# Autodesk Inventor assembly: ElectronicsHousing
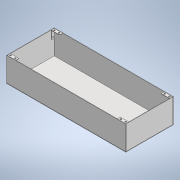
[picture p0: Inventor's stored thumbnail of the model, 180x180]
Saved by Autodesk Inventor 2020 (Build 240168000, 168)
## iProperties
Created: 2021-11-12
Part Number: ElectronicsHousing
Document SubType Name: Assembly
Designer: 17185
Author: 17185
## Documents named in this file (3)
- C:\Users\17185\Desktop\chassis draft\ElectronicsHousing\ElectronicsHousing.iam
- C:\Users\17185\Desktop\chassis draft\ElectronicsHousing\ElectronicsCasing.iam
- C:\Users\17185\Desktop\chassis draft\CornerBrace.ipt
## Components (5 placed, 2 different names)
1. ElectronicsCasing:1 [sub-assembly] — Mate:1, Mate:2, Flush:2, Mate:3, Mate:4, Mate:5, Mate:6, Mate:7, Flush:4, Mate:8
2. CornerBrace:1 — Flush:3, Mate:7, Mate:8
3. CornerBrace:2 — Mate:5, Mate:6, Flush:3, Flush:4
4. CornerBrace:3 — Mate:2, Flush:1, Flush:2, Mate:4
5. CornerBrace:4 — Mate:1, Flush:1, Mate:3
## Relationships (12: Mate 8, Flush 4)
- Mate:1: ElectronicsCasing:1 ↔ CornerBrace:4
- Mate:2: ElectronicsCasing:1 ↔ CornerBrace:3
- Flush:1: CornerBrace:3 ↔ CornerBrace:4
- Flush:2: ElectronicsCasing:1 ↔ CornerBrace:3
- Mate:3: ElectronicsCasing:1 ↔ CornerBrace:4
- Mate:4: ElectronicsCasing:1 ↔ CornerBrace:3
- Mate:5: ElectronicsCasing:1 ↔ CornerBrace:2
- Mate:6: ElectronicsCasing:1 ↔ CornerBrace:2
- Flush:3: CornerBrace:1 ↔ CornerBrace:2
- Mate:7: ElectronicsCasing:1 ↔ CornerBrace:1
- Flush:4: ElectronicsCasing:1 ↔ CornerBrace:2
- Mate:8: ElectronicsCasing:1 ↔ CornerBrace:1
